# Autodesk Inventor assembly: LeapMotionArm_v1.0
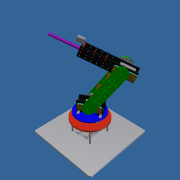
[picture p0: Inventor's stored thumbnail of the model, 180x180]
Saved by Autodesk Inventor 2012 (Build 160160000, 160)
## iProperties
Created: 2014-03-29
Part Number: LeapMotionArm_v1.0
Document SubType Name: Assembly
Designer: Admin
Author: Admin
## Documents named in this file (25)
- C:\Users\Admin\Documents\Inventor\LeapMotionArm\LeapMotionArm_v1.0.iam
- C:\Users\Admin\Documents\Inventor\LeapMotionArm\ServoFutabaS3003.ipt
- C:\Users\Admin\Documents\Inventor\LeapMotionArm\ServoFutabaS3003_circularArm.ipt
- C:\Users\Admin\Documents\Inventor\LeapMotionArm\Acrylic_rotationServoMount.ipt
- C:\Users\Admin\Documents\Inventor\LeapMotionArm\StandOff_2.0inch.ipt
- C:\Users\Admin\Documents\Inventor\LeapMotionArm\Acrylic_rotationServoTray.ipt
- C:\Users\Admin\Documents\Inventor\LeapMotionArm\LowerArm.ipt
- C:\Users\Admin\Documents\Inventor\LeapMotionArm\LowerArm_Support.ipt
- C:\Users\Admin\Documents\Inventor\LeapMotionArm\Acrylic_YawServoSupport_1.ipt
- C:\Users\Admin\Documents\Inventor\LeapMotionArm\LCouplerSmall.ipt
- C:\Users\Admin\Documents\Inventor\LeapMotionArm\Acrylic_YawServoSupport_2.ipt
- C:\Users\Admin\Documents\Inventor\LeapMotionArm\Acrylic_YawServoSupport_3.ipt
- C:\Users\Admin\Documents\Inventor\LeapMotionArm\Acrylic_YawServoSupport_4.ipt
- C:\Users\Admin\Documents\Inventor\LeapMotionArm\ServoFutabaS3003_UpperArm.ipt
- C:\Users\Admin\Documents\Inventor\LeapMotionArm\Acrylic_UpperArm.ipt
- C:\Users\Admin\Documents\Inventor\LeapMotionArm\Acrylic_UpperArm_Support.ipt
- C:\Users\Admin\Documents\Inventor\LeapMotionArm\Acrylic_PitchServoSupport_1.ipt
- C:\Users\Admin\Documents\Inventor\LeapMotionArm\Acrylic_PitchServoSupport_2.ipt
- C:\Users\Admin\Documents\Inventor\LeapMotionArm\Acrylic_2.2_LowerArmBridge.ipt
- C:\Users\Admin\Documents\Inventor\LeapMotionArm\Acrylic_2.2_UpperArmBridge.ipt
- C:\Users\Admin\Documents\Inventor\LeapMotionArm\CatFeather.ipt
- C:\Users\Admin\Documents\Inventor\LeapMotionArm\Acrylic_2.2_UpperArmBridge_cameraMount.ipt
- C:\Users\Admin\Documents\Inventor\LeapMotionArm\Acrylic_5.8_cameraMount.ipt
- C:\Users\Admin\Documents\Inventor\LeapMotionArm\Acrylic_6_Base.ipt
- C:\Users\Admin\Documents\Inventor\LeapMotionArm\arduino uno.iam
## Components (39 placed, 24 different names)
1. ServoFutabaS3003:1 — Mate:1, Flush:1, Mate:3, Angle:1, Mate:12, Mate:27, Mate:49
2. ServoFutabaS3003_circularArm:1 — Mate:1, Flush:1, Mate:13, Mate:14
3. Acrylic_5.8_rotationServoMount:1 — Mate:3, Angle:1, Mate:4, Mate:5, Mate:6, Mate:7, Mate:8, Mate:9, Mate:10, Mate:11, Angle:2, Angle:3, Mate:49
4. StandOff_2.0inch:1 — Mate:4, Mate:8, Tangent:2, Tangent:3
5. StandOff_2.0inch:2 — Mate:6, Mate:10
6. StandOff_2.0inch:3 — Mate:5, Mate:11
7. StandOff_2.0inch:4 — Mate:7, Mate:9, Mate:89, Tangent:4
8. Acrylic_2.8_rotationServoTray:1 — Mate:12, Mate:13, Mate:14, Angle:2, Mate:24, Mate:26, Angle:6, Mate:30, Mate:33, Mate:34, Mate:35, Mate:36
9. ServoFutabaS3003:2 — Mate:15, Flush:2, Angle:3, Mate:18, Angle:5, Mate:25, Mate:26, Angle:6, Mate:27, Flush:3, Flush:5
10. ServoFutabaS3003_circularArm:2 — Mate:15, Flush:2, Mate:21, Mate:22
11. LowerArm:1 — Mate:18, Mate:19, Mate:20, Mate:21, Mate:22, Mate:46, Mate:47, Mate:55, Mate:56, Mate:80
12. LowerArm_Support:1 — Mate:19, Mate:20, Mate:44, Mate:54, Mate:57, Mate:61, Mate:62, Mate:63, Mate:64, Mate:65, Mate:66, Mate:67, Mate:68, Mate:69
13. Acrylic_YawServoSupport_1:1 — Angle:5, Mate:24, Mate:25, Flush:3, Mate:31, Mate:32, Flush:4, Flush:6, Flush:7
14. LCouplerSmall:1 — Mate:32, Mate:33, Flush:6
15. LCouplerSmall:2 — Mate:30, Mate:31, Flush:7
16. Acrylic_YawServoSupport_2:1 — Mate:34, Flush:4, Flush:5, Mate:37, Mate:38, Flush:8, Flush:9, Mate:39, Angle:7, Mate:40, Flush:10
17. LCouplerSmall:3 — Mate:36, Mate:37, Flush:8
18. LCouplerSmall:4 — Mate:35, Mate:38, Flush:9
19. Acrylic_YawServoSupport_3:1 — Mate:39, Angle:7, Mate:40, Flush:10, Mate:41, Mate:42, Mate:43
20. Acrylic_YawServoSupport_4:1 — Mate:41, Mate:42, Mate:43, Mate:44
21. ServoFutabaS3003_UpperArm:1 — Mate:45, Flush:11, Mate:46, Mate:48, Angle:8, Flush:12, Flush:13, Flush:16
22. ServoFutabaS3003_circularArm:3 — Mate:45, Flush:11, Mate:47, Mate:80
23. Acrylic_UpperArm:1 — Mate:48, Angle:8, Flush:12, Flush:13, Flush:14, Flush:15, Mate:73, Mate:74, Mate:75, Mate:76, Mate:77, Mate:78
24. Acrylic_UpperArm_Support:1 — Flush:14, Flush:15, Flush:16, Flush:17, Mate:50, Flush:18, Mate:81, Mate:82, Mate:83
25. Acrylic_PitchServoSupport_1:1 — Flush:17, Mate:50, Flush:18, Mate:51, Mate:52, Mate:53
26. Acrylic_PitchServoSupport_2:1 — Mate:51, Mate:52, Mate:53, Mate:54
27. Acrylic_2.2_LowerArmBridge:1 — Mate:55, Mate:56, Mate:57
28. Acrylic_2.2_LowerArmBridge:2 — Mate:67, Mate:68, Mate:69
29. Acrylic_2.2_LowerArmBridge:3 — Mate:61, Mate:62, Mate:63
30. Acrylic_2.2_LowerArmBridge:4 — Mate:64, Mate:65, Mate:66
31. Acrylic_2.2_UpperArmBridge:2 — Mate:73, Mate:74, Mate:75
32. Acrylic_2.2_UpperArmBridge:3 — Mate:76, Mate:77, Mate:78, Flush:19
33. CatFeather:1 — Flush:19
34. Acrylic_2.2_UpperArmBridge_cameraMount:1 — Mate:81, Mate:82, Mate:83, Mate:84, Mate:85, Angle:9
35. LCouplerSmall:5 — Mate:84, Mate:85, Angle:9, Mate:87, Mate:88
36. Acrylic_5.8_cameraMount:1 — Mate:86, Flush:20, Flush:21, Mate:87, Mate:88
37. Acrylic_5.8_cameraMount:2 — Mate:86, Flush:20, Flush:21
38. Acrylic_6_Base:1 — Mate:89, Tangent:2, Tangent:3, Tangent:4, Mate:90, Angle:10, Flush:22, Flush:23
39. arduino uno:1 [sub-assembly] — Mate:90, Angle:10, Flush:22, Flush:23
## Relationships (112: Mate 77, Flush 23, Angle 9, Tangent 3)
- Mate:1: ServoFutabaS3003:1 ↔ ServoFutabaS3003_circularArm:1
- Flush:1: ServoFutabaS3003:1 ↔ ServoFutabaS3003_circularArm:1
- Mate:3: ServoFutabaS3003:1 ↔ Acrylic_5.8_rotationServoMount:1
- Angle:1 (0 deg): ServoFutabaS3003:1 ↔ Acrylic_5.8_rotationServoMount:1
- Mate:4: Acrylic_5.8_rotationServoMount:1 ↔ StandOff_2.0inch:1
- Mate:5: Acrylic_5.8_rotationServoMount:1 ↔ StandOff_2.0inch:3
- Mate:6: Acrylic_5.8_rotationServoMount:1 ↔ StandOff_2.0inch:2
- Mate:7: Acrylic_5.8_rotationServoMount:1 ↔ StandOff_2.0inch:4
- Mate:8: Acrylic_5.8_rotationServoMount:1 ↔ StandOff_2.0inch:1
- Mate:9: Acrylic_5.8_rotationServoMount:1 ↔ StandOff_2.0inch:4
- Mate:10: Acrylic_5.8_rotationServoMount:1 ↔ StandOff_2.0inch:2
- Mate:11: Acrylic_5.8_rotationServoMount:1 ↔ StandOff_2.0inch:3
- Mate:12: ServoFutabaS3003:1 ↔ Acrylic_2.8_rotationServoTray:1
- Mate:13: ServoFutabaS3003_circularArm:1 ↔ Acrylic_2.8_rotationServoTray:1
- Mate:14: ServoFutabaS3003_circularArm:1 ↔ Acrylic_2.8_rotationServoTray:1
- Angle:2 (0 deg): Acrylic_5.8_rotationServoMount:1 ↔ Acrylic_2.8_rotationServoTray:1
- Mate:15: ServoFutabaS3003:2 ↔ ServoFutabaS3003_circularArm:2
- Flush:2: ServoFutabaS3003:2 ↔ ServoFutabaS3003_circularArm:2
- Angle:3 (0 deg): Acrylic_5.8_rotationServoMount:1 ↔ ServoFutabaS3003:2
- Mate:18: ServoFutabaS3003:2 ↔ LowerArm:1
- Mate:19: LowerArm:1 ↔ LowerArm_Support:1
- Mate:20: LowerArm:1 ↔ LowerArm_Support:1
- Mate:21: ServoFutabaS3003_circularArm:2 ↔ LowerArm:1
- Mate:22: ServoFutabaS3003_circularArm:2 ↔ LowerArm:1
- Angle:5 (0 deg): ServoFutabaS3003:2 ↔ Acrylic_YawServoSupport_1:1
- Mate:24: Acrylic_2.8_rotationServoTray:1 ↔ Acrylic_YawServoSupport_1:1
- Mate:25: ServoFutabaS3003:2 ↔ Acrylic_YawServoSupport_1:1
- Mate:26 (10 mm): Acrylic_2.8_rotationServoTray:1 ↔ ServoFutabaS3003:2
- Angle:6 (0 deg): Acrylic_2.8_rotationServoTray:1 ↔ ServoFutabaS3003:2
- Mate:27: ServoFutabaS3003:1 ↔ ServoFutabaS3003:2
- Flush:3 (4.75 mm): ServoFutabaS3003:2 ↔ Acrylic_YawServoSupport_1:1
- Mate:30: Acrylic_2.8_rotationServoTray:1 ↔ LCouplerSmall:2
- Mate:31: Acrylic_YawServoSupport_1:1 ↔ LCouplerSmall:2
- Mate:32: Acrylic_YawServoSupport_1:1 ↔ LCouplerSmall:1
- Mate:33: Acrylic_2.8_rotationServoTray:1 ↔ LCouplerSmall:1
- Mate:34: Acrylic_2.8_rotationServoTray:1 ↔ Acrylic_YawServoSupport_2:1
- Flush:4: Acrylic_YawServoSupport_1:1 ↔ Acrylic_YawServoSupport_2:1
- Flush:5: ServoFutabaS3003:2 ↔ Acrylic_YawServoSupport_2:1
- Flush:6 (3 mm): Acrylic_YawServoSupport_1:1 ↔ LCouplerSmall:1
- Flush:7 (3 mm): Acrylic_YawServoSupport_1:1 ↔ LCouplerSmall:2
- Mate:35: Acrylic_2.8_rotationServoTray:1 ↔ LCouplerSmall:4
- Mate:36: Acrylic_2.8_rotationServoTray:1 ↔ LCouplerSmall:3
- Mate:37: Acrylic_YawServoSupport_2:1 ↔ LCouplerSmall:3
- Mate:38: Acrylic_YawServoSupport_2:1 ↔ LCouplerSmall:4
- Flush:8 (3 mm): Acrylic_YawServoSupport_2:1 ↔ LCouplerSmall:3
- Flush:9 (3 mm): Acrylic_YawServoSupport_2:1 ↔ LCouplerSmall:4
- Mate:39: Acrylic_YawServoSupport_2:1 ↔ Acrylic_YawServoSupport_3:1
- Angle:7 (0 deg): Acrylic_YawServoSupport_2:1 ↔ Acrylic_YawServoSupport_3:1
- Mate:40: Acrylic_YawServoSupport_2:1 ↔ Acrylic_YawServoSupport_3:1
- Flush:10 (2.5 mm): Acrylic_YawServoSupport_2:1 ↔ Acrylic_YawServoSupport_3:1
- Mate:41: Acrylic_YawServoSupport_3:1 ↔ Acrylic_YawServoSupport_4:1
- Mate:42: Acrylic_YawServoSupport_3:1 ↔ Acrylic_YawServoSupport_4:1
- Mate:43: Acrylic_YawServoSupport_3:1 ↔ Acrylic_YawServoSupport_4:1
- Mate:44: LowerArm_Support:1 ↔ Acrylic_YawServoSupport_4:1
- Mate:45: ServoFutabaS3003_UpperArm:1 ↔ ServoFutabaS3003_circularArm:3
- Flush:11: ServoFutabaS3003_UpperArm:1 ↔ ServoFutabaS3003_circularArm:3
- Mate:46: LowerArm:1 ↔ ServoFutabaS3003_UpperArm:1
- Mate:47: LowerArm:1 ↔ ServoFutabaS3003_circularArm:3
- Mate:48: ServoFutabaS3003_UpperArm:1 ↔ Acrylic_UpperArm:1
- Angle:8 (0 deg): ServoFutabaS3003_UpperArm:1 ↔ Acrylic_UpperArm:1
- Flush:12: ServoFutabaS3003_UpperArm:1 ↔ Acrylic_UpperArm:1
- Flush:13 (-5.1 mm): ServoFutabaS3003_UpperArm:1 ↔ Acrylic_UpperArm:1
- Mate:49: ServoFutabaS3003:1 ↔ Acrylic_5.8_rotationServoMount:1
- Flush:14: Acrylic_UpperArm:1 ↔ Acrylic_UpperArm_Support:1
- Flush:15: Acrylic_UpperArm:1 ↔ Acrylic_UpperArm_Support:1
- Flush:16: ServoFutabaS3003_UpperArm:1 ↔ Acrylic_UpperArm_Support:1
- Flush:17: Acrylic_UpperArm_Support:1 ↔ Acrylic_PitchServoSupport_1:1
- Mate:50: Acrylic_UpperArm_Support:1 ↔ Acrylic_PitchServoSupport_1:1
- Flush:18 (5 mm): Acrylic_UpperArm_Support:1 ↔ Acrylic_PitchServoSupport_1:1
- Mate:51: Acrylic_PitchServoSupport_1:1 ↔ Acrylic_PitchServoSupport_2:1
- Mate:52: Acrylic_PitchServoSupport_1:1 ↔ Acrylic_PitchServoSupport_2:1
- Mate:53: Acrylic_PitchServoSupport_1:1 ↔ Acrylic_PitchServoSupport_2:1
- Mate:54: LowerArm_Support:1 ↔ Acrylic_PitchServoSupport_2:1
- Mate:55: LowerArm:1 ↔ Acrylic_2.2_LowerArmBridge:1
- Mate:56: LowerArm:1 ↔ Acrylic_2.2_LowerArmBridge:1
- Mate:57: LowerArm_Support:1 ↔ Acrylic_2.2_LowerArmBridge:1
- Mate:61: LowerArm_Support:1 ↔ Acrylic_2.2_LowerArmBridge:3
- Mate:62: LowerArm_Support:1 ↔ Acrylic_2.2_LowerArmBridge:3
- Mate:63: LowerArm_Support:1 ↔ Acrylic_2.2_LowerArmBridge:3
- Mate:64: LowerArm_Support:1 ↔ Acrylic_2.2_LowerArmBridge:4
- Mate:65: LowerArm_Support:1 ↔ Acrylic_2.2_LowerArmBridge:4
- Mate:66: LowerArm_Support:1 ↔ Acrylic_2.2_LowerArmBridge:4
- Mate:67: LowerArm_Support:1 ↔ Acrylic_2.2_LowerArmBridge:2
- Mate:68: LowerArm_Support:1 ↔ Acrylic_2.2_LowerArmBridge:2
- Mate:69: LowerArm_Support:1 ↔ Acrylic_2.2_LowerArmBridge:2
- Mate:73 (-0.5 mm): Acrylic_UpperArm:1 ↔ Acrylic_2.2_UpperArmBridge:2
- Mate:74: Acrylic_UpperArm:1 ↔ Acrylic_2.2_UpperArmBridge:2
- Mate:75: Acrylic_UpperArm:1 ↔ Acrylic_2.2_UpperArmBridge:2
- Mate:76 (-0.5 mm): Acrylic_UpperArm:1 ↔ Acrylic_2.2_UpperArmBridge:3
- Mate:77: Acrylic_UpperArm:1 ↔ Acrylic_2.2_UpperArmBridge:3
- Mate:78: Acrylic_UpperArm:1 ↔ Acrylic_2.2_UpperArmBridge:3
- Flush:19: Acrylic_2.2_UpperArmBridge:3 ↔ CatFeather:1
- Mate:80: LowerArm:1 ↔ ServoFutabaS3003_circularArm:3
- Mate:81 (-0.5 mm): Acrylic_UpperArm_Support:1 ↔ Acrylic_2.2_UpperArmBridge_cameraMount:1
- Mate:82: Acrylic_UpperArm_Support:1 ↔ Acrylic_2.2_UpperArmBridge_cameraMount:1
- Mate:83: Acrylic_UpperArm_Support:1 ↔ Acrylic_2.2_UpperArmBridge_cameraMount:1
- Mate:84: Acrylic_2.2_UpperArmBridge_cameraMount:1 ↔ LCouplerSmall:5
- Mate:85: Acrylic_2.2_UpperArmBridge_cameraMount:1 ↔ LCouplerSmall:5
- Angle:9 (0 deg): Acrylic_2.2_UpperArmBridge_cameraMount:1 ↔ LCouplerSmall:5
- Mate:86: Acrylic_5.8_cameraMount:1 ↔ Acrylic_5.8_cameraMount:2
- Flush:20: Acrylic_5.8_cameraMount:1 ↔ Acrylic_5.8_cameraMount:2
- Flush:21: Acrylic_5.8_cameraMount:1 ↔ Acrylic_5.8_cameraMount:2
- Mate:87: LCouplerSmall:5 ↔ Acrylic_5.8_cameraMount:1
- Mate:88: LCouplerSmall:5 ↔ Acrylic_5.8_cameraMount:1
- Mate:89: StandOff_2.0inch:4 ↔ Acrylic_6_Base:1
- Tangent:2 (-82.645 mm): StandOff_2.0inch:1 ↔ Acrylic_6_Base:1
- Tangent:3 (-82.645 mm): StandOff_2.0inch:1 ↔ Acrylic_6_Base:1
- Tangent:4 (-82.645 mm): StandOff_2.0inch:4 ↔ Acrylic_6_Base:1
- Mate:90 (4.8 mm): Acrylic_6_Base:1 ↔ arduino uno:1
- Angle:10 (0 deg): Acrylic_6_Base:1 ↔ arduino uno:1
- Flush:22 (80.75 mm): Acrylic_6_Base:1 ↔ arduino uno:1
- Flush:23 (88.33 mm): Acrylic_6_Base:1 ↔ arduino uno:1
